# Autodesk Inventor assembly: roller assembly
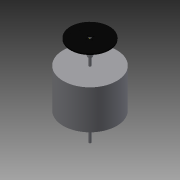
[picture p0: Inventor's stored thumbnail of the model, 180x180]
Saved by Autodesk Inventor 2015 (Build 190159000, 159)
## iProperties
Created: 2014-11-08
Part Number: roller assembly
Document SubType Name: Assembly
Designer: jesse
Author: jesse
## Documents named in this file (6)
- C:\Users\jesse\Desktop\robot\arm\roller assembly.iam
- C:\Users\jesse\Desktop\robot\arm\foam gripper2.ipt
- C:\Users\jesse\Desktop\robot\arm\roller.ipt
- C:\Users\jesse\Desktop\robot\arm\rotating rod.ipt
- C:\Users\jesse\Desktop\robot\stock parts\hub_motor_shaft_2012\hub_motor_shaft_2012.ipt
- C:\Users\jesse\Desktop\robot\arm\adaptor.ipt
## Components (5 placed, 5 different names)
1. foam gripper2:1 — Mate:2, Mate:3, Mate:4, Mate:5
2. roller:1 — Mate:2
3. rotating rod:1 — Mate:3, Mate:8
4. hub_motor_shaft_2012:1 — Mate:4, Mate:5, Mate:6, Mate:7
5. adaptor:1 — Mate:6, Mate:7, Mate:8
## Relationships (7: Mate 7)
- Mate:2: foam gripper2:1 ↔ roller:1
- Mate:3: foam gripper2:1 ↔ rotating rod:1
- Mate:4: foam gripper2:1 ↔ hub_motor_shaft_2012:1
- Mate:5: foam gripper2:1 ↔ hub_motor_shaft_2012:1
- Mate:6: hub_motor_shaft_2012:1 ↔ adaptor:1
- Mate:7: hub_motor_shaft_2012:1 ↔ adaptor:1
- Mate:8: rotating rod:1 ↔ adaptor:1
